# Autodesk Inventor assembly: Montagem_v2
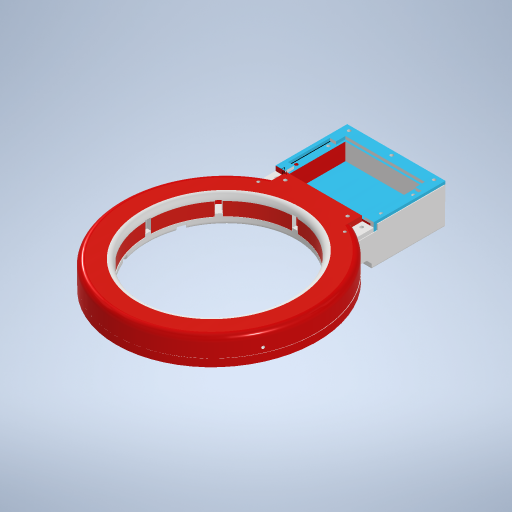
[picture p0: Inventor's stored thumbnail of the model, 512x512]
Saved by Autodesk Inventor 2024.3 (Build 283343000, 343)
## iProperties
Created: 2025-02-20
Part Number: Montagem_v2
Document SubType Name: Assembly
Designer: lostv
Author: lostv
## Documents named in this file (6)
- C:\Users\lostv\OneDrive\Área de Trabalho\Organizacao_Pesquisa\modelos_3D_IPT\Montagem_v2.iam
- C:\Users\lostv\OneDrive\Área de Trabalho\Organizacao_Pesquisa\modelos_3D_IPT\anel_v2.ipt
- C:\Users\lostv\OneDrive\Área de Trabalho\Organizacao_Pesquisa\modelos_3D_IPT\peca_principal_v2.ipt
- C:\Users\lostv\OneDrive\Área de Trabalho\Organizacao_Pesquisa\modelos_3D_IPT\tampa_anel_v2.ipt
- C:\Users\lostv\OneDrive\Área de Trabalho\Organizacao_Pesquisa\modelos_3D_IPT\suporte_lcd_botoes.ipt
- C:\Users\lostv\OneDrive\Área de Trabalho\Organizacao_Pesquisa\modelos_3D_IPT\tampa_principal_v2.ipt
## Components (5 placed, 5 different names)
1. anel_v2:1
2. peca_principal_v2:1
3. tampa_anel_v2:1
4. suporte_lcd_botoes:1
5. tampa_principal_v2:1
## Named parameters: Finish1_Area = 563.823, Finish2_Area = 68.7573, Finish3_Area = 270.42, Finish4_Area = 363.658
note: some values were not read from the file. Shown as the stored number, unit unknown: "Finish1_Area", "Finish2_Area", "Finish3_Area", "Finish4_Area".
